# Autodesk Inventor assembly: Monitor Mount
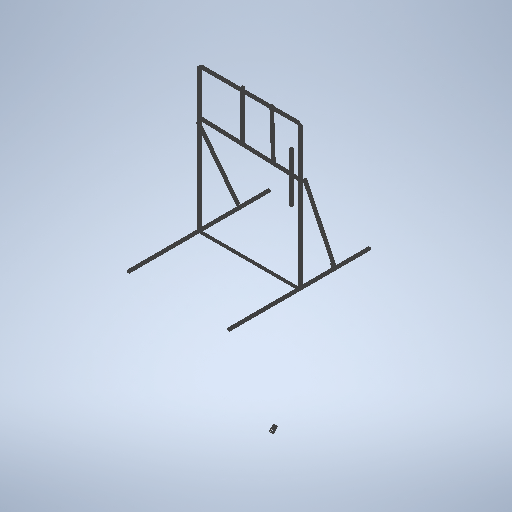
[picture p0: Inventor's stored thumbnail of the model, 512x512]
Saved by Autodesk Inventor 2027 (Build 310192000, 192)
## iProperties
Created: 2026-05-19
Part Number: Monitor Mount
Document SubType Name: Assembly
Designer: IG2
Author: IG2
## Documents named in this file (7)
- C:\Users\ig2\Desktop\SMR Thermal\thermal-loop\resources\CAD_models\V0.1\Inventor\.iam files\Monitor Mount.iam
- C:\Users\ig2\Desktop\SMR Thermal\thermal-loop\resources\CAD_models\V0.1\Inventor\.ipt files\T-Slotted Framing Inline Pivotfor 1_inch Single Rail.ipt
- C:\Users\ig2\Desktop\SMR Thermal\thermal-loop\resources\CAD_models\V0.1\Inventor\.ipt files\60 inch T-Slotted Framing Rail.ipt
- C:\Users\ig2\Desktop\SMR Thermal\thermal-loop\resources\CAD_models\V0.1\Inventor\.ipt files\25.4 inch T-Slotted Framing Rail.ipt
- C:\Users\ig2\Desktop\SMR Thermal\thermal-loop\resources\CAD_models\V0.1\Inventor\.ipt files\T-Slotted Framing Inline Pivotfor 1_inch Single Rail_MIR.ipt
- C:\Users\ig2\Desktop\SMR Thermal\thermal-loop\resources\CAD_models\V0.1\Inventor\.ipt files\72 inch T-Slotted Framing Rail.ipt
- C:\Users\ig2\Desktop\SMR Thermal\thermal-loop\resources\CAD_models\V0.1\Inventor\.ipt files\50 inch T-Slotted Framing Rail.ipt
## Components (15 placed, 6 different names)
1. T-Slotted Framing Inline Pivotfor 1_inch Single Rail:2 — Rigid:3
2. T-Slotted Framing Inline Pivotfor 1_inch Single Rail:1 — Rigid:2
3. 60 inch T-Slotted Framing Rail:1
4. 60 inch T-Slotted Framing Rail:2 — Rigid:1
5. 25.4 inch T-Slotted Framing Rail:1
6. 25.4 inch T-Slotted Framing Rail:2
7. 25.4 inch T-Slotted Framing Rail:3
8. T-Slotted Framing Inline Pivotfor 1_inch Single Rail_MIR:1
9. 72 inch T-Slotted Framing Rail:1 — Rigid:1
10. 72 inch T-Slotted Framing Rail:2
11. 72 inch T-Slotted Framing Rail:3 — Mate:1
12. 72 inch T-Slotted Framing Rail:4
13. 50 inch T-Slotted Framing Rail:1 — Rigid:3
14. 50 inch T-Slotted Framing Rail:2 — Rigid:2
15. 60 inch T-Slotted Framing Rail:3 — Mate:1
## Relationships (4: WeldJoint 3, Mate 1)
- Rigid:1 [WeldJoint] (7.62 mm): 60 inch T-Slotted Framing Rail:2 ↔ 72 inch T-Slotted Framing Rail:1
- Rigid:2 [WeldJoint]: T-Slotted Framing Inline Pivotfor 1_inch Single Rail:1 ↔ 50 inch T-Slotted Framing Rail:2
- Mate:1: 72 inch T-Slotted Framing Rail:3 ↔ 60 inch T-Slotted Framing Rail:3
- Rigid:3 [WeldJoint]: T-Slotted Framing Inline Pivotfor 1_inch Single Rail:2 ↔ 50 inch T-Slotted Framing Rail:1
